# Autodesk Inventor assembly: 810001-X1
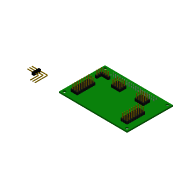
[picture p0: Inventor's stored thumbnail of the model, 180x180]
Saved by Autodesk Inventor 2015 (Build 190159000, 159)
## iProperties
Created: 2013-01-19
Part Number: 810001-X1
Document SubType Name: Assembly
Designer: davidgitz
Author: davidgitz
## Documents named in this file (5)
- C:\SharedDrive\Dropbox\FAST Robotics\Products\810001_FAST Robot Shield\CAD\810001_FAST Robot Shield\810001-X1.iam
- C:\SharedDrive\Dropbox\FAST Robotics\Products\810001_FAST Robot Shield\CAD\810001_FAST Robot Shield\MainBoard.ipt
- C:\SharedDrive\Dropbox\FAST Robotics\Products\810001_FAST Robot Shield\CAD\810001_FAST Robot Shield\Header1x1.ipt
- C:\SharedDrive\Dropbox\FAST Robotics\Products\811000_Parallax Quickstart\CAD\811000_Parallax Quickstart\702871018.ipt
- C:\SharedDrive\Dropbox\FAST Robotics\Products\810001_FAST Robot Shield\CAD\810001_FAST Robot Shield\HeaderRight3.ipt
## Components (81 placed, 4 different names)
1. MainBoard:1 — Mate:2, Mate:3, Mate:4, Mate:5, Mate:6, Mate:7, Angle:1, Angle:2, Flush:7, Flush:8, Flush:9, Flush:10, Mate:9, Flush:12, Flush:13
2. 702871018:1 — Mate:9, Flush:12, Flush:13
3. HeaderRight3:1
4. Header1x1:1
5. Header1x1:2
6. Header1x1:3
7. Header1x1:4
8. Header1x1:5
9. Header1x1:6
10. Header1x1:7
11. Header1x1:8
12. Header1x1:9
13. Header1x1:10 — Flush:6
14. Header1x1:11
15. Header1x1:12 — Mate:6, Flush:4
16. Header1x1:17
17. Header1x1:58
18. Header1x1:59
19. Header1x1:60
20. Header1x1:61
21. Header1x1:62
22. Header1x1:63
23. Header1x1:64
24. Header1x1:65 — Flush:4, Flush:7
25. Header1x1:66
26. Header1x1:67 — Mate:2
27. Header1x1:68
28. Header1x1:15 — Flush:5
29. Header1x1:69
30. Header1x1:70
31. Header1x1:71 — Flush:9
32. Header1x1:72
33. Header1x1:73
34. Header1x1:74
35. Header1x1:75
36. Header1x1:76
37. Header1x1:77 — Mate:3
38. Header1x1:78
39. Header1x1:79
40. Header1x1:80
41. Header1x1:81
42. Header1x1:82
43. Header1x1:83
44. Header1x1:84
45. Header1x1:85
46. Header1x1:86 — Angle:2
47. Header1x1:87
48. Header1x1:88
49. Header1x1:89
50. Header1x1:90
51. Header1x1:91
52. Header1x1:14 — Mate:5, Flush:3
53. Header1x1:92 — Mate:8, Flush:6
54. Header1x1:93
55. Header1x1:94
56. Header1x1:16 — Flush:11
57. Header1x1:95
58. Header1x1:96
59. Header1x1:97
60. Header1x1:98 — Flush:10
61. Header1x1:99
62. Header1x1:100
63. Header1x1:101
64. Header1x1:102
65. Header1x1:103
66. Header1x1:104
67. Header1x1:105
68. Header1x1:106
69. Header1x1:107
70. Header1x1:108 — Mate:4
71. Header1x1:109 — Flush:8
72. Header1x1:110
73. Header1x1:111
74. Header1x1:112 — Angle:1
75. Header1x1:113
76. Header1x1:114
77. Header1x1:115
78. Header1x1:116
79. Header1x1:117 — Flush:5
80. Header1x1:18 — Mate:7
81. Header1x1:118 — Flush:3, Mate:8, Flush:11
## Component patterns: Ultrasonic:4x3 (12 elements), Servo:4x3 (12 elements), ADC:4x3 (24 elements), ToAPM:4x1 (4 elements), GPIO:8x3 (24 elements), HighPower:2x1 (2 elements)
## Relationships (21: Flush 11, Mate 8, Angle 2)
- Mate:2: MainBoard:1 ↔ Header1x1:67
- Mate:3: MainBoard:1 ↔ Header1x1:77
- Mate:4: MainBoard:1 ↔ Header1x1:108
- Mate:5: MainBoard:1 ↔ Header1x1:14
- Mate:6: MainBoard:1 ↔ Header1x1:12
- Mate:7: MainBoard:1 ↔ Header1x1:18
- Flush:3: Header1x1:14 ↔ Header1x1:118
- Mate:8: Header1x1:92 ↔ Header1x1:118
- Flush:4: Header1x1:12 ↔ Header1x1:65
- Angle:1 (0 deg): MainBoard:1 ↔ Header1x1:112
- Angle:2 (0 deg): MainBoard:1 ↔ Header1x1:86
- Flush:5: Header1x1:15 ↔ Header1x1:117
- Flush:6: Header1x1:10 ↔ Header1x1:92
- Flush:7 (10.16 mm): MainBoard:1 ↔ Header1x1:65
- Flush:8 (6.35 mm): MainBoard:1 ↔ Header1x1:109
- Flush:9 (6.35 mm): MainBoard:1 ↔ Header1x1:71
- Flush:10 (6.35 mm): MainBoard:1 ↔ Header1x1:98
- Flush:11: Header1x1:16 ↔ Header1x1:118
- Mate:9: MainBoard:1 ↔ 702871018:1
- Flush:12 (3.048 mm): MainBoard:1 ↔ 702871018:1
- Flush:13 (12.446 mm): MainBoard:1 ↔ 702871018:1
